# Autodesk Inventor assembly: full_rack
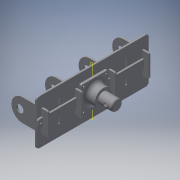
[picture p0: Inventor's stored thumbnail of the model, 180x180]
Saved by Autodesk Inventor 2016 (Build 200138000, 138)
## iProperties
Created: 2018-10-08
Part Number: full_rack
Document SubType Name: Assembly
Designer: andrew
Author: andrew
## Documents named in this file (5)
- C:\Users\andre\OneDrive\Uni_Work\Bench_corrosion_motor\Sample_rack\full_rack.iam
- C:\Users\andre\OneDrive\Uni_Work\Bench_corrosion_motor\Sample_rack\sample_mount.ipt
- C:\Users\andre\OneDrive\Uni_Work\Bench_corrosion_motor\Sample_rack\mounting_plate.ipt
- C:\Users\andre\OneDrive\Uni_Work\Bench_corrosion_motor\Sample_rack\pin.ipt
- C:\Users\andre\OneDrive\Uni_Work\Bench_corrosion_motor\Sample_rack\adaptor.ipt
## Components (7 placed, 4 different names)
1. mounting_plate:1 — Rigid:1, Rotational:1, Rotational:2
2. pin:1 — Rotational:1
3. adaptor:1 — Rotational:2
4. sample_mount:1 — Rigid:1
5. sample_mount:2
6. sample_mount:3
7. sample_mount:4
## Component patterns: (4 elements, first: sample_mount:1)
## Relationships (3: RevoluteJoint 2, WeldJoint 1)
- Rigid:1 [WeldJoint]: mounting_plate:1 ↔ sample_mount:1
- Rotational:1 [RevoluteJoint]: mounting_plate:1 ↔ pin:1
- Rotational:2 [RevoluteJoint]: mounting_plate:1 ↔ adaptor:1
